# Autodesk Inventor assembly: HS 36T Gear, Circle_mirrored
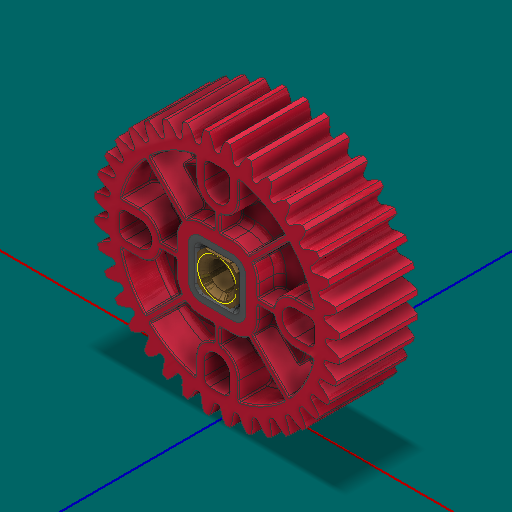
[picture p0: Inventor's stored thumbnail of the model, 512x512]
Saved by Autodesk Inventor 2025 (Build 290162000, 162)
## iProperties
Created: 2022-08-02
Part Number: HS 36T Gear, Circle_mirrored
Document SubType Name: Assembly
Designer: averey
Author: ylu12
## Documents named in this file (3)
- C:\Users\avere\vex_robotics_high_stakes\hardware\cad\ATLAS\chassis\drive_pod\back_left\gearbox\HS 36T Gear, Circle_mirrored.iam
- C:\Users\avere\vex_robotics_high_stakes\hardware\cad\ATLAS\chassis\drive_pod\back_left\gearbox\HS Shaft Adapter Circle_mirrored.ipt
- C:\Users\avere\vex_robotics_high_stakes\hardware\cad\ATLAS\chassis\drive_pod\back_left\gearbox\HS 36T Gear, No Insert_mirrored.ipt
## Components (2 placed, 2 different names)
1. HS Shaft Adapter Circle_mirrored:1 — Flush:1, Mate:2, Mate:1
2. HS 36T Gear, No Insert_mirrored:1 — Mate:10, Mate:9, Flush:5
## Relationships (6: Mate 4, Flush 2)
- Flush:1 (-6.35 mm): HS Shaft Adapter Circle_mirrored:1
- Mate:2: HS Shaft Adapter Circle_mirrored:1
- Mate:1: HS Shaft Adapter Circle_mirrored:1
- Mate:10: HS 36T Gear, No Insert_mirrored:1
- Mate:9: HS 36T Gear, No Insert_mirrored:1
- Flush:5: HS 36T Gear, No Insert_mirrored:1
